# Autodesk Inventor assembly: Servo motor
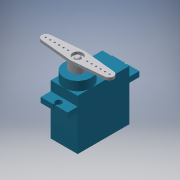
[picture p0: Inventor's stored thumbnail of the model, 180x180]
Saved by Autodesk Inventor 2018 (Build 220112000, 112)
## iProperties
Created: 2018-06-25
Part Number: Servo motor
Document SubType Name: Assembly
Designer: Ajith Thomas
Author: Ajith Thomas
## Documents named in this file (3)
- C:\Users\Ajith Thomas\Dropbox\Gas_Sensing_Robot\FumeBot-Design\Servo motor\Servo motor.iam
- C:\Users\Ajith Thomas\Dropbox\Gas_Sensing_Robot\FumeBot-Design\Servo motor\Servo body.ipt
- C:\Users\Ajith Thomas\Dropbox\Gas_Sensing_Robot\FumeBot-Design\Servo motor\Servo shaft and horn.ipt
## Components (2 placed, 2 different names)
1. Servo body:1 — Mate:1, Mate:2, Servo drive
2. Servo shaft and horn:1 — Mate:1, Mate:2, Servo drive
## Relationships (3: Mate 2, Angle 1)
- Mate:1: Servo body:1 ↔ Servo shaft and horn:1
- Mate:2: Servo body:1 ↔ Servo shaft and horn:1
- Servo drive [Angle] (0 deg): Servo body:1 ↔ Servo shaft and horn:1
